# Autodesk Inventor assembly: Wenkel_GoleaCristian
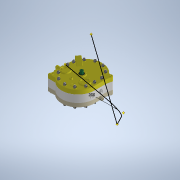
[picture p0: Inventor's stored thumbnail of the model, 180x180]
Saved by Autodesk Inventor 2021 (Build 250183000, 183)
## iProperties
Created: 2021-04-08
Part Number: Wenkel_GoleaCristian
Document SubType Name: Assembly
Designer: Crist
Unghi: 0,00 deg
Author: Crist
## Documents named in this file (10)
- C:\Users\Crist\Desktop\Facultate\CAD\#Proiecte\Animatie_Golea Cristian\Wenkel_GoleaCristian.iam
- C:\Users\Crist\Desktop\Facultate\CAD\#Proiecte\Animatie_Golea Cristian\CapacSpate.ipt
- C:\Users\Crist\Desktop\Facultate\CAD\#Proiecte\Animatie_Golea Cristian\StatorWankel.ipt
- C:\Users\Crist\Desktop\Facultate\CAD\#Proiecte\Animatie_Golea Cristian\Arbore.ipt
- C:\Users\Crist\Desktop\Facultate\CAD\#Proiecte\Animatie_Golea Cristian\SansRotor.iam
- C:\Users\Crist\Desktop\Facultate\CAD\#Proiecte\Animatie_Golea Cristian\SansCapacFata.iam
- C:\Users\Crist\Desktop\Facultate\CAD\#Proiecte\Animatie_Golea Cristian\Ans Suruburi Fixare.iam
- C:\Users\Crist\Desktop\Facultate\CAD\#Proiecte\Animatie_Golea Cristian\Ans Piulite Fixare.iam
- C:\Users\Crist\Documents\Inventor\Content Center Files\R2021\en-US\ISO 6194 1  T 1\ISO 6194_1 - Type1 22 x 35 x 7.ipt
- C:\Users\Crist\Desktop\Facultate\CAD\#Proiecte\Wankel_GoleaCristian\Traseu.ipt
## Components (10 placed, 9 different names)
1. CapacSpate:1 — Mate:1, Mate:2, Angle:1, Mate:3, Mate:4, Mate:5, Mate:10
2. StatorWankel:1 — Mate:1, Mate:2, Angle:1, Unghi animatie, Mate:7, Mate:9
3. Arbore:1 — Mate:3, Mate:4, Unghi animatie, Mate:6, Angle:3, Rotation:1, Mate:8, Mate:11, Mate:13
4. SansRotor:1 [sub-assembly] — Mate:5, Mate:6, Angle:3, Rotation:1
5. SansCapacFata:1 [sub-assembly] — Mate:7, Mate:8, Mate:9, Mate:12
6. Ans Suruburi Fixare:1 [sub-assembly]
7. Ans Piulite Fixare:1 [sub-assembly]
8. ISO 6194/1 Type 1 Type1 22 x 35 x 7:1 — Mate:10, Mate:11
9. ISO 6194/1 Type 1 Type1 22 x 35 x 7:2 — Mate:12, Mate:13
10. Traseu:1 — Flush:1
## Relationships (20: Mate 13, Angle 3, Insert 2, RelateRotation 1, Flush 1)
- Mate:1: CapacSpate:1 ↔ StatorWankel:1
- Mate:2: CapacSpate:1 ↔ StatorWankel:1
- Angle:1 (0 deg): CapacSpate:1 ↔ StatorWankel:1
- Mate:3 (1 mm): CapacSpate:1 ↔ Arbore:1
- Mate:4: CapacSpate:1 ↔ Arbore:1
- Unghi animatie [Angle] (0 deg): StatorWankel:1 ↔ Arbore:1
- Mate:5: CapacSpate:1 ↔ SansRotor:1
- Mate:6: Arbore:1 ↔ SansRotor:1
- Angle:3 (0 deg): Arbore:1 ↔ SansRotor:1
- Rotation:1 [RelateRotation] (3 ul): Arbore:1 ↔ SansRotor:1
- Mate:7: StatorWankel:1 ↔ SansCapacFata:1
- Mate:8: Arbore:1 ↔ SansCapacFata:1
- Mate:9: StatorWankel:1 ↔ SansCapacFata:1
- [Insert]: SansCapacFata:1 ↔ Ans Suruburi Fixare:1
- [Insert]: CapacSpate:1 ↔ Ans Piulite Fixare:1
- Mate:10: CapacSpate:1 ↔ ISO 6194/1 Type 1 Type1 22 x 35 x 7:1
- Mate:11: Arbore:1 ↔ ISO 6194/1 Type 1 Type1 22 x 35 x 7:1
- Mate:12: SansCapacFata:1 ↔ ISO 6194/1 Type 1 Type1 22 x 35 x 7:2
- Mate:13: Arbore:1 ↔ ISO 6194/1 Type 1 Type1 22 x 35 x 7:2
- Flush:1: Traseu:1
